# Autodesk Inventor assembly: 머리 조립품
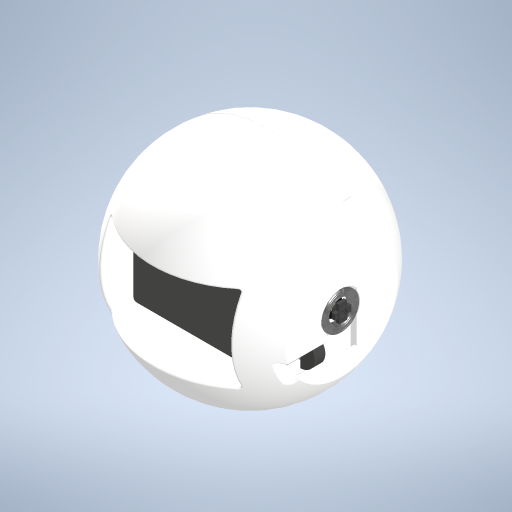
[picture p0: Inventor's stored thumbnail of the model, 512x512]
Saved by Autodesk Inventor 2023.1 (Build 271208000, 208)
## iProperties
Created: 2022-08-09
Part Number: 머리 조립품
Document SubType Name: Assembly
Designer: fly01
Author: fly01
## Documents named in this file (10)
- C:\Users\fly01\Desktop\PAI설계 2\조림품\머리 조립품.iam
- C:\Users\fly01\Desktop\PAI설계 2\출력품\Head_front.ipt
- C:\Users\fly01\Desktop\PAI설계 2\조림품\라즈베리파이 조립품.iam
- C:\Users\fly01\Desktop\PAI설계 2\출력품\라즈베리파이 고정 커버.ipt
- C:\Users\fly01\Desktop\PAI설계 2\범용 부품\쿨러.ipt
- C:\Users\fly01\Desktop\PAI설계 2\출력품\Head_back.ipt
- C:\Users\fly01\Desktop\PAI설계 2\범용 부품\180도 서보모터.ipt
- C:\Users\fly01\Desktop\PAI설계 2\범용 부품\베어링 6802zz.ipt
- C:\Users\fly01\Desktop\PAI설계 2\범용 부품\베어링 MR84ZZ.ipt
- C:\Users\fly01\Desktop\PAI설계 2\범용 부품\180도 서보모터 십자축 자른 것.ipt
## Components (9 placed, 9 different names)
1. Head_front:1 — 삽입:1, 삽입:2, 삽입:3, 플러쉬:1, 삽입:5, 회전:2, 삽입:8, 삽입:9
2. 라즈베리파이 조립품:1 [sub-assembly] — 회전:1
3. 라즈베리파이 고정 커버:1 — 회전:1, 삽입:1, 삽입:2
4. 쿨러:1 — 회전:2
5. Head_back:1 — 삽입:3
6. 180도 서보모터:1 — 플러쉬:1, 삽입:7, 삽입:8
7. 베어링 6802zz:1 — 삽입:5
8. 베어링 MR84ZZ:1 — 삽입:9
9. 180도 서보모터 십자축 자른 것:1 — 삽입:7
## Relationships (10: Insert 7, RevoluteJoint 2, Flush 1)
- 회전:1 [RevoluteJoint]: 라즈베리파이 조립품:1 ↔ 라즈베리파이 고정 커버:1
- 삽입:1 [Insert]: Head_front:1 ↔ 라즈베리파이 고정 커버:1
- 삽입:2 [Insert]: Head_front:1 ↔ 라즈베리파이 고정 커버:1
- 삽입:3 [Insert]: Head_front:1 ↔ Head_back:1
- 플러쉬:1 [Flush]: Head_front:1 ↔ 180도 서보모터:1
- 삽입:5 [Insert]: Head_front:1 ↔ 베어링 6802zz:1
- 회전:2 [RevoluteJoint]: Head_front:1 ↔ 쿨러:1
- 삽입:7 [Insert]: 180도 서보모터:1 ↔ 180도 서보모터 십자축 자른 것:1
- 삽입:8 [Insert]: Head_front:1 ↔ 180도 서보모터:1
- 삽입:9 [Insert]: Head_front:1 ↔ 베어링 MR84ZZ:1
